# Autodesk Inventor assembly: ASY SLM 0100 frame
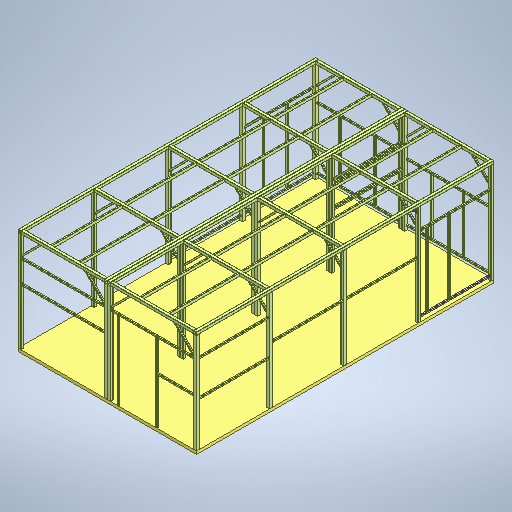
[picture p0: Inventor's stored thumbnail of the model, 512x512]
Saved by Autodesk Inventor 2025.4 (Build 294407000, 407)
## iProperties
Created: 2025-12-15
Part Number: ASY SLM 0100 frame
Document SubType Name: Assembly
Designer: admin
Mass: 1.42177e+07 g
Surface Area: 6.18137e+06 cm^2
Volume: 9.68441e+06 cm^3
Density: 1.4681 g/cm^3
Author: admin
## Documents named in this file (26)
- C:\Users\admin\Documents\Inventor\SLM-Salemal\ASY SLM 0100 frame.iam
- C:\Users\admin\Documents\Inventor\SLM-Salemal\ASY SLM 1600 Filter column D940.iam
- C:\Users\admin\Documents\Inventor\SLM-Salemal\Оборудование Инвентор\HY-H H2162–4T.ipt
- C:\Users\admin\Documents\Inventor\SLM-Salemal\Оборудование Инвентор\UV-Cleaner ODV-15.ipt
- C:\Users\admin\Documents\Inventor\SLM-Salemal\Оборудование Инвентор\Станции дозирования\Coagulant barrel.ipt
- C:\Users\admin\Documents\Inventor\SLM-Salemal\Оборудование Инвентор\Станции дозирования\Flocculant barrel.ipt
- C:\Users\admin\Documents\Inventor\SLM-Salemal\Оборудование Инвентор\Станции дозирования\GPHN barrel.ipt
- C:\Users\admin\Documents\Inventor\SLM-Salemal\Оборудование Инвентор\Станции дозирования\Soda barrel.ipt
- C:\Users\admin\Documents\Inventor\SLM-Salemal\Оборудование Инвентор\Вертикальный насос\CDM(F)15-4 FSWP(S_L)C\CDM(F)15-4 FSWP(S_L)C.iam
- C:\Users\admin\Documents\Inventor\SLM-Salemal\Оборудование Инвентор\Вертикальный насос\CDM(F)65-2-2 FSWP(S)C\CDM(F)65-2-2 FSWP(S)C.iam
- C:\Users\admin\Documents\Inventor\SLM-Salemal\ASY SLM 1110 MAIN FRAME.iam
- C:\Users\admin\Documents\Inventor\SLM-Salemal\ASY SLM 1210 MAIN FRAME.iam
- C:\Users\admin\Documents\Inventor\SLM-Salemal\Оборудование Инвентор\Electrical box 1.ipt
- C:\Users\admin\Documents\Inventor\SLM-Salemal\Оборудование Инвентор\Electrical box 2.ipt
- C:\Users\admin\Documents\Inventor\SLM-Salemal\Оборудование Инвентор\Electrical box 3.ipt
- C:\Users\admin\Documents\Inventor\SLM-Salemal\Оборудование Инвентор\Electrical box 4.ipt
- C:\Users\admin\Documents\Inventor\SLM-Salemal\roof frame\ASY SLM 1300 frame roof.iam
- C:\Users\admin\Documents\Inventor\SLM-Salemal\ISO 4019 - 80x80x3 - 8000.ipt
- C:\Users\admin\Documents\Inventor\SLM-Salemal\Cyclone\Гидроциклон.ipt
- C:\Users\admin\Documents\Inventor\SLM-Salemal\pump frame1\ASY SLM-1810 pump pillar.iam
- C:\Users\admin\Documents\Inventor\SLM-Salemal\pump frame2\Workspaces\Workspace\ASY SLM-1820 pump frame.iam
- C:\Users\admin\Documents\Inventor\SLM-Salemal\SLM- -Sandwich roof.ipt
- C:\Users\admin\Documents\Inventor\SLM-Salemal\SLM- -Sandwich wall low.ipt
- C:\Users\admin\Documents\Inventor\SLM-Salemal\SLM- -Sandwich wall.ipt
- C:\Users\admin\Documents\Inventor\SLM-Salemal\Оборудование Инвентор\Pipe clamp bracket.ipt
- C:\Users\admin\Documents\Inventor\SLM-Salemal\SLM- Floordummy.ipt
## Components (48 placed, 25 different names)
1. HY-H H2162–4T:1 — Flush:28, Mate:17
2. UV-Cleaner ODV-15:1
3. Coagulant barrel:1 — Flush:29
4. Flocculant barrel:1 — Flush:31
5. GPHN barrel:1 — Flush:29, Flush:30, Flush:31, Mate:18
6. Soda barrel:1 — Flush:30
7. CDM(F)65-2-2 FSWP(S)C:1 [sub-assembly]
8. HY-H H2162–4T:2 — Flush:28
9. CDM(F)15-4 FSWP(S_L)C:2 [sub-assembly]
10. CDM(F)65-2-2 FSWP(S)C:2 [sub-assembly]
11. UV-Cleaner ODV-15:2
12. ASY SLM 1110 FLOOR FRAME:1 [sub-assembly] — Mate:12, Mate:13, Flush:14, Flush:15, Mate:14, Flush:22, Flush:23, Mate:15, Flush:25, Mate:17, Mate:18, Mate:19, Mate:21, Mate:23, Mate:25, Mate:29, Mate:31, Mate:32, Flush:35, Flush:42, Mate:42, Mate:43, Mate:44, Flush:46, Flush:47, Flush:48, Flush:49, Flush:50
13. ASY SLM 1210 MAIN FRAME:1 [sub-assembly] — Flush:26, Mate:16, Flush:27, Mate:20, Mate:22, Mate:24, Mate:26, Mate:28, Mate:30, Flush:32, Flush:33, Mate:35, Flush:36, Mate:36, Flush:43, Mate:41, Flush:44, Flush:52, Flush:53
14. CDM(F)15-4 FSWP(S_L)C:5 [sub-assembly]
15. ASY SLM 1600 Filter column D940:24 [sub-assembly] — Flush:2, Flush:3, Flush:4, Flush:5, Flush:9, Flush:10, Flush:11, Mate:13, Flush:14, Flush:15
16. ASY SLM 1600 Filter column D940:20 [sub-assembly] — Flush:2, Flush:3, Flush:11, Flush:12
17. ASY SLM 1600 Filter column D940:26 [sub-assembly] — Flush:4, Flush:9, Flush:12, Flush:13
18. ASY SLM 1600 Filter column D940:23 [sub-assembly] — Flush:5, Flush:10, Flush:13, Mate:12
19. ASY SLM 1600 Filter column D940:27 [sub-assembly]
20. ASY SLM 1600 Filter column D940:28 [sub-assembly] — Mate:14, Flush:22
21. ASY SLM 1600 Filter column D940:29 [sub-assembly] — Flush:23
22. Electrical box 1:1 — Mate:19, Mate:20
23. Electrical box 2:1 — Mate:28, Mate:29
24. Electrical box 3:1 — Mate:25, Mate:26
25. Electrical box 4:1 — Mate:23, Mate:24
26. Electrical box 4:2 — Mate:21, Mate:22
27. ASY SLM 1300 frame roof:1 [sub-assembly] — Rigid:2, Rigid:3
28. ASY SLM 1300 frame roof:2 [sub-assembly] — Rigid:3, Rigid:4
29. ASY SLM 1300 frame roof:3 [sub-assembly] — Mate:30, Flush:32, Flush:33, Rigid:1, Rigid:6, Rigid:7, Rigid:8, Rigid:9, Rigid:10
30. ASY SLM 1300 frame roof:4 [sub-assembly] — Rigid:1, Rigid:2
31. ASY SLM 1300 frame roof:5 [sub-assembly] — Rigid:4, Flush:37, Mate:38, Flush:41, Mate:39
32. ISO 4019 - 80x80x3 - 8000:1 — Mate:38, Flush:41, Mate:39
33. ISO 4019 - 80x80x3 - 8000:2 — Rigid:6, Mate:34
34. ISO 4019 - 80x80x3 - 8000:3 — Rigid:7
35. ISO 4019 - 80x80x3 - 8000:4 — Rigid:8, Mate:37
36. ISO 4019 - 80x80x3 - 8000:5 — Rigid:9, Flush:39
37. ISO 4019 - 80x80x3 - 8000:6 — Rigid:10
38. Гидроциклон:1 — Mate:43, Flush:48, Flush:49
39. ASY SLM-1810 pump pillar:1 [sub-assembly] — Mate:32
40. ASY SLM-1820 pump frame:1 [sub-assembly] — Flush:50
41. SLM- -Sandwich roof:1 — Mate:34, Flush:37, Flush:40, Mate:40
42. SLM- -Sandwich wall low:1 — Mate:35, Flush:35, Flush:36, Mate:40
43. SLM- -Sandwich wall:1 — Mate:36, Flush:42, Flush:43
44. SLM- -Sandwich roof:2 — Mate:37, Flush:39, Flush:40
45. Pipe clamp bracket:1 — Mate:41, Flush:44
46. Pipe clamp bracket:2 — Mate:42
47. Гидроциклон:2 — Mate:44, Flush:46, Flush:47
48. SLM- Floordummy:1 — Flush:51, Flush:52, Flush:53
## Relationships (85: Flush 45, Mate 31, WeldJoint 9)
- Flush:2: ASY SLM 1600 Filter column D940:24 ↔ ASY SLM 1600 Filter column D940:20
- Flush:3: ASY SLM 1600 Filter column D940:24 ↔ ASY SLM 1600 Filter column D940:20
- Flush:4: ASY SLM 1600 Filter column D940:24 ↔ ASY SLM 1600 Filter column D940:26
- Flush:5: ASY SLM 1600 Filter column D940:24 ↔ ASY SLM 1600 Filter column D940:23
- Flush:9: ASY SLM 1600 Filter column D940:24 ↔ ASY SLM 1600 Filter column D940:26
- Flush:10: ASY SLM 1600 Filter column D940:24 ↔ ASY SLM 1600 Filter column D940:23
- Flush:11 (-1100 mm): ASY SLM 1600 Filter column D940:24 ↔ ASY SLM 1600 Filter column D940:20
- Flush:12 (-1100 mm): ASY SLM 1600 Filter column D940:20 ↔ ASY SLM 1600 Filter column D940:26
- Flush:13 (1100 mm): ASY SLM 1600 Filter column D940:26 ↔ ASY SLM 1600 Filter column D940:23
- Mate:12 (3 mm): ASY SLM 1110 FLOOR FRAME:1 ↔ ASY SLM 1600 Filter column D940:23
- Mate:13: ASY SLM 1110 FLOOR FRAME:1 ↔ ASY SLM 1600 Filter column D940:24
- Flush:14 (100 mm): ASY SLM 1110 FLOOR FRAME:1 ↔ ASY SLM 1600 Filter column D940:24
- Flush:15: ASY SLM 1110 FLOOR FRAME:1 ↔ ASY SLM 1600 Filter column D940:24
- [Flush]: ASY SLM 1600 Filter column D940:27 ↔ ASY SLM 1600 Filter column D940:28
- [Flush]: ASY SLM 1600 Filter column D940:27 ↔ ASY SLM 1600 Filter column D940:28
- [Flush]: ASY SLM 1600 Filter column D940:28 ↔ ASY SLM 1600 Filter column D940:29
- [Flush]: ASY SLM 1600 Filter column D940:28 ↔ ASY SLM 1600 Filter column D940:29
- [Flush] (-1100 mm): ASY SLM 1600 Filter column D940:27 ↔ ASY SLM 1600 Filter column D940:28
- [Flush] (-1100 mm): ASY SLM 1600 Filter column D940:27 ↔ ASY SLM 1600 Filter column D940:29
- Mate:14: ASY SLM 1110 FLOOR FRAME:1 ↔ ASY SLM 1600 Filter column D940:28
- Flush:22 (100 mm): ASY SLM 1110 FLOOR FRAME:1 ↔ ASY SLM 1600 Filter column D940:28
- Flush:23 (2375 mm): ASY SLM 1110 FLOOR FRAME:1 ↔ ASY SLM 1600 Filter column D940:29
- Mate:15: ASY SLM 1110 FLOOR FRAME:1
- Flush:25: ASY SLM 1110 FLOOR FRAME:1
- Flush:26: ASY SLM 1210 MAIN FRAME:1
- Mate:16: ASY SLM 1210 MAIN FRAME:1
- Flush:27: ASY SLM 1210 MAIN FRAME:1
- Flush:28: HY-H H2162–4T:1 ↔ HY-H H2162–4T:2
- Mate:17: HY-H H2162–4T:1 ↔ ASY SLM 1110 FLOOR FRAME:1
- Flush:29: Coagulant barrel:1 ↔ GPHN barrel:1
- Flush:30: GPHN barrel:1 ↔ Soda barrel:1
- Flush:31: Flocculant barrel:1 ↔ GPHN barrel:1
- Mate:18: GPHN barrel:1 ↔ ASY SLM 1110 FLOOR FRAME:1
- Mate:19 (1400 mm): ASY SLM 1110 FLOOR FRAME:1 ↔ Electrical box 1:1
- Mate:20: ASY SLM 1210 MAIN FRAME:1 ↔ Electrical box 1:1
- Mate:21: ASY SLM 1110 FLOOR FRAME:1 ↔ Electrical box 4:2
- Mate:22: ASY SLM 1210 MAIN FRAME:1 ↔ Electrical box 4:2
- Mate:23: ASY SLM 1110 FLOOR FRAME:1 ↔ Electrical box 4:1
- Mate:24: ASY SLM 1210 MAIN FRAME:1 ↔ Electrical box 4:1
- Mate:25 (1500 mm): ASY SLM 1110 FLOOR FRAME:1 ↔ Electrical box 3:1
- Mate:26: ASY SLM 1210 MAIN FRAME:1 ↔ Electrical box 3:1
- Mate:28: ASY SLM 1210 MAIN FRAME:1 ↔ Electrical box 2:1
- Mate:29 (1500 mm): ASY SLM 1110 FLOOR FRAME:1 ↔ Electrical box 2:1
- Mate:30: ASY SLM 1210 MAIN FRAME:1 ↔ ASY SLM 1300 frame roof:3
- Flush:32: ASY SLM 1210 MAIN FRAME:1 ↔ ASY SLM 1300 frame roof:3
- Flush:33: ASY SLM 1210 MAIN FRAME:1 ↔ ASY SLM 1300 frame roof:3
- Rigid:1 [WeldJoint] (-1980 mm): ASY SLM 1300 frame roof:3 ↔ ASY SLM 1300 frame roof:4
- Rigid:2 [WeldJoint] (-2000 mm): ASY SLM 1300 frame roof:1 ↔ ASY SLM 1300 frame roof:4
- Rigid:3 [WeldJoint] (-2000 mm): ASY SLM 1300 frame roof:1 ↔ ASY SLM 1300 frame roof:2
- Rigid:4 [WeldJoint] (-1980 mm): ASY SLM 1300 frame roof:2 ↔ ASY SLM 1300 frame roof:5
- Rigid:6 [WeldJoint]: ASY SLM 1300 frame roof:3 ↔ ISO 4019 - 80x80x3 - 8000:2
- Rigid:7 [WeldJoint]: ASY SLM 1300 frame roof:3 ↔ ISO 4019 - 80x80x3 - 8000:3
- Rigid:8 [WeldJoint]: ASY SLM 1300 frame roof:3 ↔ ISO 4019 - 80x80x3 - 8000:4
- Rigid:9 [WeldJoint]: ASY SLM 1300 frame roof:3 ↔ ISO 4019 - 80x80x3 - 8000:5
- Rigid:10 [WeldJoint]: ASY SLM 1300 frame roof:3 ↔ ISO 4019 - 80x80x3 - 8000:6
- Mate:31: ASY SLM 1110 FLOOR FRAME:1
- Mate:32: ASY SLM 1110 FLOOR FRAME:1 ↔ ASY SLM-1810 pump pillar:1
- Mate:34: ISO 4019 - 80x80x3 - 8000:2 ↔ SLM- -Sandwich roof:1
- Mate:35: ASY SLM 1210 MAIN FRAME:1 ↔ SLM- -Sandwich wall low:1
- Flush:35 (20 mm): ASY SLM 1110 FLOOR FRAME:1 ↔ SLM- -Sandwich wall low:1
- Flush:36 (-100 mm): ASY SLM 1210 MAIN FRAME:1 ↔ SLM- -Sandwich wall low:1
- Flush:37 (-200 mm): ASY SLM 1300 frame roof:5 ↔ SLM- -Sandwich roof:1
- Mate:36: ASY SLM 1210 MAIN FRAME:1 ↔ SLM- -Sandwich wall:1
- Mate:37: ISO 4019 - 80x80x3 - 8000:4 ↔ SLM- -Sandwich roof:2
- Flush:39 (-177 mm): ISO 4019 - 80x80x3 - 8000:5 ↔ SLM- -Sandwich roof:2
- Flush:40: SLM- -Sandwich roof:1 ↔ SLM- -Sandwich roof:2
- Mate:38: ASY SLM 1300 frame roof:5 ↔ ISO 4019 - 80x80x3 - 8000:1
- Flush:41: ASY SLM 1300 frame roof:5 ↔ ISO 4019 - 80x80x3 - 8000:1
- Mate:39 (-5 mm): ASY SLM 1300 frame roof:5 ↔ ISO 4019 - 80x80x3 - 8000:1
- Mate:40 (100 mm): SLM- -Sandwich roof:1 ↔ SLM- -Sandwich wall low:1
- Flush:42 (21 mm): ASY SLM 1110 FLOOR FRAME:1 ↔ SLM- -Sandwich wall:1
- Flush:43: ASY SLM 1210 MAIN FRAME:1 ↔ SLM- -Sandwich wall:1
- Mate:41: ASY SLM 1210 MAIN FRAME:1 ↔ Pipe clamp bracket:1
- Flush:44: ASY SLM 1210 MAIN FRAME:1 ↔ Pipe clamp bracket:1
- Mate:42: ASY SLM 1110 FLOOR FRAME:1 ↔ Pipe clamp bracket:2
- Mate:43 (280 mm): ASY SLM 1110 FLOOR FRAME:1 ↔ Гидроциклон:1
- Mate:44 (550 mm): ASY SLM 1110 FLOOR FRAME:1 ↔ Гидроциклон:2
- Flush:46 (550 mm): ASY SLM 1110 FLOOR FRAME:1 ↔ Гидроциклон:2
- Flush:47 (350 mm): ASY SLM 1110 FLOOR FRAME:1 ↔ Гидроциклон:2
- Flush:48 (650 mm): ASY SLM 1110 FLOOR FRAME:1 ↔ Гидроциклон:1
- Flush:49 (350 mm): ASY SLM 1110 FLOOR FRAME:1 ↔ Гидроциклон:1
- Flush:50 (205 mm): ASY SLM 1110 FLOOR FRAME:1 ↔ ASY SLM-1820 pump frame:1
- Flush:51: SLM- Floordummy:1
- Flush:52: ASY SLM 1210 MAIN FRAME:1 ↔ SLM- Floordummy:1
- Flush:53: ASY SLM 1210 MAIN FRAME:1 ↔ SLM- Floordummy:1
## Named parameters: d70_d50 = 0 mm, d71_d52 = 0 mm, d72_d53 = 0 mm, d73_d58 = 0 mm, d74_d60 = -1100 mm, d75_d61 = -1100 mm
